# Autodesk Inventor assembly: Сборка12
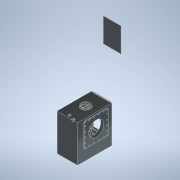
[picture p0: Inventor's stored thumbnail of the model, 180x180]
Saved by Autodesk Inventor 2021 (Build 250183000, 183)
## iProperties
Created: 2020-12-06
Part Number: Сборка12
Document SubType Name: Assembly
Designer: Тимоха
Author: Тимоха
## Documents named in this file (10)
- C:\Users\Тимоха\Desktop\КР Компрессор\compressor\Сборка12.iam
- C:\Users\Тимоха\Desktop\КР Компрессор\compressor\Картер.ipt
- C:\Users\Тимоха\Desktop\КР Компрессор\compressor\Балка.ipt
- C:\Users\Тимоха\Desktop\КР Компрессор\compressor\Крышка стенки картера низ.ipt
- C:\Users\Тимоха\Desktop\КР Компрессор\compressor\Нижняя часть коренного подшипника.ipt
- C:\Users\Тимоха\Desktop\КР Компрессор\compressor\Крышка стенки картера верх.ipt
- C:\Users\Тимоха\Desktop\КР Компрессор\compressor\Крышка коренного подшипника1.ipt
- C:\Users\Тимоха\Desktop\КР Компрессор\compressor\Крышка картера 1.ipt
- C:\Users\Тимоха\Desktop\КР Компрессор\compressor\Крышка картера 2.ipt
- C:\Users\Тимоха\Desktop\КР Компрессор\compressor\Крышка картера 3.ipt
## Components (14 placed, 9 different names)
1. Картер:1 — Жесткий:5, Жесткий:6, Жесткий:7, Жесткий:9, Жесткий:12
2. Балка:1 — Жесткий:5
3. Балка:2 — Жесткий:6
4. Крышка стенки картера низ:1 — Жесткий:9, Жесткий:10
5. Нижняя часть коренного подшипника:1
6. Нижняя часть коренного подшипника:2
7. Нижняя часть коренного подшипника:3 — Жесткий:8
8. Крышка стенки картера верх:1 — Жесткий:10, Жесткий:11
9. Крышка коренного подшипника1:1
10. Нижняя часть коренного подшипника:4
11. Крышка картера 1:1 — Жесткий:11
12. Крышка картера 2:1
13. Крышка картера 3:1 — Жесткий:12
14. Крышка коренного подшипника1:2 — Жесткий:7, Жесткий:8
## Relationships (22: WeldJoint 12, Flush 10)
- [Flush]: Картер:1 ↔ Крышка стенки картера низ:1
- [Flush]: Картер:1 ↔ Крышка стенки картера низ:1
- [WeldJoint]: Картер:1 ↔ Нижняя часть коренного подшипника:1
- [WeldJoint]: Картер:1 ↔ Нижняя часть коренного подшипника:2
- [Flush]: Картер:1 ↔ Крышка стенки картера верх:1
- [Flush]: Картер:1 ↔ Крышка стенки картера верх:1
- [WeldJoint]: Нижняя часть коренного подшипника:2 ↔ Нижняя часть коренного подшипника:4
- [WeldJoint]: Картер:1 ↔ Крышка коренного подшипника1:1
- [Flush]: Картер:1 ↔ Крышка картера 1:1
- [Flush]: Картер:1 ↔ Крышка картера 1:1
- [Flush]: Картер:1 ↔ Крышка картера 2:1
- [Flush]: Картер:1 ↔ Крышка картера 2:1
- [Flush]: Картер:1 ↔ Крышка картера 3:1
- [Flush]: Картер:1 ↔ Крышка картера 3:1
- Жесткий:5 [WeldJoint]: Картер:1 ↔ Балка:1
- Жесткий:6 [WeldJoint]: Картер:1 ↔ Балка:2
- Жесткий:7 [WeldJoint]: Картер:1 ↔ Крышка коренного подшипника1:2
- Жесткий:8 [WeldJoint]: Нижняя часть коренного подшипника:3 ↔ Крышка коренного подшипника1:2
- Жесткий:9 [WeldJoint]: Картер:1 ↔ Крышка стенки картера низ:1
- Жесткий:10 [WeldJoint]: Крышка стенки картера низ:1 ↔ Крышка стенки картера верх:1
- Жесткий:11 [WeldJoint]: Крышка стенки картера верх:1 ↔ Крышка картера 1:1
- Жесткий:12 [WeldJoint]: Картер:1 ↔ Крышка картера 3:1
## Named parameters: d10_d11 = 0 mm, d11_d13 = 0 mm
